# Autodesk Inventor assembly: Four Fiber Bundle
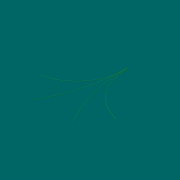
[picture p0: Inventor's stored thumbnail of the model, 180x180]
Saved by Autodesk Inventor 2016 (Build 200138000, 138)
## iProperties
Created: 2015-08-17
Part Number: Four Fiber Bundle
Document SubType Name: Assembly
Designer: Cosmic
Author: Cosmic
## Documents named in this file (4)
- C:\Users\Sawaiz\Documents\3d\inventor\ScintillatorPanel\tree\treeFiberBundle.iam
- C:\Users\Sawaiz\Documents\3d\inventor\ScintillatorPanel\tree\treeLongFiber.ipt
- C:\Users\Sawaiz\Documents\3d\inventor\ScintillatorPanel\tree\treeShortFiber.ipt
- C:\Users\Sawaiz\Documents\3d\inventor\ScintillatorPanel\Scintillator.xlsx
## Components (4 placed, 2 different names)
1. treeLongFiber:1 — Flush:2, Flush:3, Tangent:7, Angle:3, Tangent:11
2. treeLongFiber:2 — Flush:2, Angle:2, Flush:4, Tangent:9, Tangent:11, Mate:1
3. treeShortFiber:1 — Tangent:3, Flush:1, Tangent:8, Tangent:9, Tangent:10, Angle:4
4. treeShortFiber:2 — Tangent:2, Flush:1, Angle:1, Flush:3, Tangent:7, Tangent:10, Angle:4
## Relationships (16: Tangent 7, Flush 4, Angle 4, Mate 1)
- Tangent:2 (0.075 mm): treeShortFiber:2
- Tangent:3 (0.075 mm): treeShortFiber:1
- Flush:1: treeShortFiber:1 ↔ treeShortFiber:2
- Angle:1 (0 deg): treeShortFiber:2
- Flush:2: treeLongFiber:1 ↔ treeLongFiber:2
- Flush:3: treeLongFiber:1 ↔ treeShortFiber:2
- Angle:2 (0 deg): treeLongFiber:2
- Tangent:7 (0.15 mm): treeLongFiber:1 ↔ treeShortFiber:2
- Angle:3 (0 deg): treeLongFiber:1
- Tangent:8: treeShortFiber:1
- Flush:4: treeLongFiber:2
- Tangent:9 (0.15 mm): treeLongFiber:2 ↔ treeShortFiber:1
- Tangent:10 (0.15 mm): treeShortFiber:1 ↔ treeShortFiber:2
- Tangent:11 (0.15 mm): treeLongFiber:1 ↔ treeLongFiber:2
- Mate:1 (0.5 mm): treeLongFiber:2
- Angle:4 (180 deg): treeShortFiber:1 ↔ treeShortFiber:2
## Named parameters: OpticalFiberDiameter = 1 mm, ScintillatorThickness = 10 mm, OpticalFiberClearence = 0.15 mm, SmallTrackDiameter = 175 mm, LargeTrackRatio = 3, ScintillatorEdgeClearence = 3 mm, ScintillatorWidth = 145 mm, ScintillatorHeight = 145 mm, ShallowTrackDepth = 1.3 mm, MPPCClearence = 0.075 mm, MPPCSensorClearence = 1.45 mm, MPPCSensorOffsett = 2.105 mm, MPPCWidth = 5.9 mm, MPPCHeight = 6.55 mm, FiberEdgeOffsett = 5 mm, MPPCDepth = 0 mm, LongFiberAngle = 30 deg, ShortFiberAngle = 78 deg, LoopLargeTrackRatio = 1.1, LoopSmallTrackDiameter = 90 mm, FiberSensorClerence = 0.5 mm, MountingScrewOffsett = 20 mm, MountingScrewDepth = 4 mm
